# Autodesk Inventor assembly: SmallSize
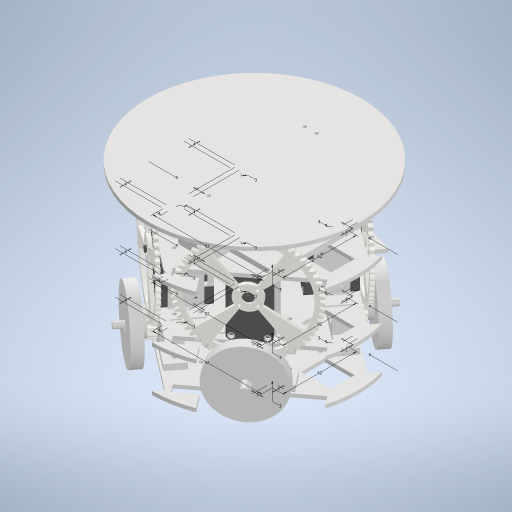
[picture p0: Inventor's stored thumbnail of the model, 512x512]
Saved by Autodesk Inventor 2023 (Build 270158000, 158)
## iProperties
Created: 2022-09-08
Part Number: SmallSize
Document SubType Name: Assembly
Designer: Lab. de Manufactura
Author: Lab. de Manufactura
## Documents named in this file (7)
- C:\Users\hiago.sodre\Downloads\SSLDynamixel\SmallSize.iam
- C:\Users\hiago.sodre\Downloads\SSLDynamixel\newbase.ipt
- C:\Users\hiago.sodre\Downloads\SSLDynamixel\soporte_eje_omni.ipt
- C:\Users\hiago.sodre\Downloads\SSLDynamixel\MotorSoporte.iam
- C:\Users\hiago.sodre\Downloads\SSLDynamixel\EjeRueda.iam
- C:\Users\hiago.sodre\Downloads\SSLDynamixel\pablo opencr.ipt
- C:\Users\hiago.sodre\Downloads\SSLDynamixel\hiago_tampassl2.ipt
## Components (17 placed, 6 different names)
1. newbase:1 — Rígido:8, Rígido:9, Rígido:10, Rígido:16
2. soporte_eje_omni:1 — Rígido:16, Rígido:17, Rígido:18
3. soporte_eje_omni:2 — Rígido:8, Rígido:19
4. soporte_eje_omni:3 — Rígido:10, Rígido:20
5. soporte_eje_omni:4 — Rígido:9, De rotación:1
6. newbase:2 — Rígido:11, Rígido:12, Rígido:13, Rígido:14, Rígido:17
7. MotorSoporte:1 [sub-assembly] — Rígido:11, Rígido:15, Rotación:4
8. MotorSoporte:2 [sub-assembly] — Rígido:14, Rotación:1
9. MotorSoporte:3 [sub-assembly] — Rígido:12, Rotación:3
10. MotorSoporte:4 [sub-assembly] — Rígido:13, Rotación:2
11. newbase:3 — Rígido:15, Mate:1
12. EjeRueda:1 [sub-assembly] — De rotación:1, Rotación:4
13. EjeRueda:2 [sub-assembly] — Rígido:18, Rotación:1
14. EjeRueda:3 [sub-assembly] — Rígido:19, Rotación:2
15. EjeRueda:4 [sub-assembly] — Rígido:20, Rotación:3
16. pablo opencr:1 — Mate:1, Mate:2
17. hiago_tampassl2:1 — Mate:2
## Relationships (20: WeldJoint 13, RelateRotation 4, Mate 2, RevoluteJoint 1)
- Rígido:8 [WeldJoint]: newbase:1 ↔ soporte_eje_omni:2
- Rígido:9 [WeldJoint]: newbase:1 ↔ soporte_eje_omni:4
- Rígido:10 [WeldJoint]: newbase:1 ↔ soporte_eje_omni:3
- Rígido:11 [WeldJoint]: newbase:2 ↔ MotorSoporte:1
- Rígido:12 [WeldJoint]: newbase:2 ↔ MotorSoporte:3
- Rígido:13 [WeldJoint]: newbase:2 ↔ MotorSoporte:4
- Rígido:14 [WeldJoint]: newbase:2 ↔ MotorSoporte:2
- Rígido:15 [WeldJoint]: MotorSoporte:1 ↔ newbase:3
- Rígido:16 [WeldJoint]: newbase:1 ↔ soporte_eje_omni:1
- Rígido:17 [WeldJoint]: soporte_eje_omni:1 ↔ newbase:2
- Rígido:18 [WeldJoint]: soporte_eje_omni:1 ↔ EjeRueda:2
- Rígido:19 [WeldJoint]: soporte_eje_omni:2 ↔ EjeRueda:3
- Rígido:20 [WeldJoint]: soporte_eje_omni:3 ↔ EjeRueda:4
- De rotación:1 [RevoluteJoint]: soporte_eje_omni:4 ↔ EjeRueda:1
- Rotación:1 [RelateRotation] (0.2 ul): MotorSoporte:2 ↔ EjeRueda:2
- Rotación:2 [RelateRotation] (0.2 ul): MotorSoporte:4 ↔ EjeRueda:3
- Rotación:3 [RelateRotation] (0.2 ul): MotorSoporte:3 ↔ EjeRueda:4
- Rotación:4 [RelateRotation] (0.2 ul): MotorSoporte:1 ↔ EjeRueda:1
- Mate:1: newbase:3 ↔ pablo opencr:1
- Mate:2: pablo opencr:1 ↔ hiago_tampassl2:1
